# Autodesk Inventor assembly: ГОРИЗОНТАЛЬНЫЙ ЗАХВАТ 1 версия
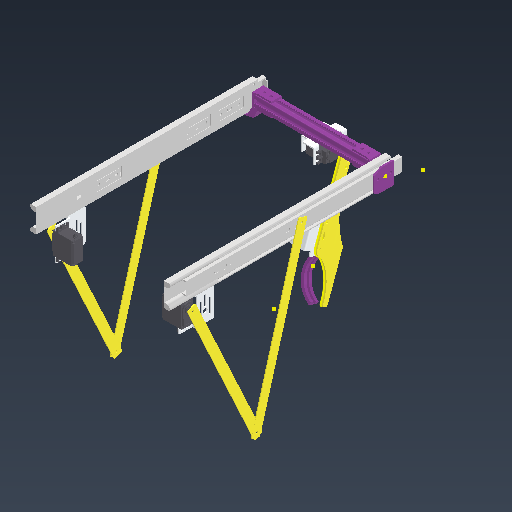
[picture p0: Inventor's stored thumbnail of the model, 512x512]
Saved by Autodesk Inventor 2025 (Build 290162000, 162)
## iProperties
Created: 2025-01-28
Part Number: ГОРИЗОНТАЛЬНЫЙ ЗАХВАТ 1 версия
Document SubType Name: Assembly
Designer: GameHD
Author: GameHD
## Documents named in this file (20)
- C:\Users\GameHD\Desktop\phantom 16950\ГОРИЗОНТАЛЬНЫЙ ЗАХВАТ 1 версия.iam
- C:\Users\GameHD\Desktop\phantom 16950\40 направляшка.iam
- C:\Users\GameHD\Desktop\phantom 16950\39070_TXM-288mm Flat Bar\39070_TXM-288mm Flat Bar.ipt
- C:\Users\GameHD\Desktop\phantom 16950\39280_txm-adjustableservobrackets\39280_txm-adjustableservobrackets.ipt
- C:\Users\GameHD\Desktop\phantom 16950\2000-0025-0002\2000-0025-0002.ipt
- C:\Users\GameHD\Desktop\phantom 16950\39070_TXM-288mm Flat Bar\длинная палка.ipt
- C:\Users\GameHD\Desktop\phantom 16950\39070_TXM-288mm Flat Bar\39070_TXM-288mm Flat Bar_MIR.ipt
- C:\Users\GameHD\Desktop\phantom 16950\39280_txm-adjustableservobrackets\39280_txm-adjustableservobrackets_MIR.ipt
- C:\Users\GameHD\Desktop\phantom 16950\2000-0025-0002\2000-0025-0002_MIR.ipt
- C:\Users\GameHD\Desktop\phantom 16950\39070_TXM-288mm Flat Bar\длинная палка_MIR.ipt
- C:\Users\GameHD\Desktop\phantom 16950\МЕЖДУ НАПРАВЛЯШКАМИ.ipt
- C:\Users\GameHD\Desktop\phantom 16950\39060_txm-standard servo bracket\39060_txm-standard servo bracket_MIR1.ipt
- C:\Users\GameHD\Desktop\phantom 16950\2000-0025-0002\2000-0025-0002_MIR2.ipt
- C:\Users\GameHD\Desktop\phantom 16950\DS3225_MG_metal_horn\DS3225_MG_metal_horn_MIR1.ipt
- C:\Users\GameHD\Desktop\phantom 16950\клешня сос_MIR1_MIR.ipt
- C:\Users\GameHD\Desktop\phantom 16950\39060_txm-standard servo bracket\39060_txm-standard servo bracket_MIR1_MIR.ipt
- C:\Users\GameHD\Desktop\phantom 16950\2000-0025-0002\2000-0025-0002_MIR2_MIR.ipt
- C:\Users\GameHD\Desktop\phantom 16950\Клешни с фиксатором\Клешни с фиксатором_MIR_MIR1_MIR.ipt
- C:\Users\GameHD\Desktop\phantom 16950\уголок п образный\уголок п образный.ipt
- C:\Users\GameHD\Desktop\phantom 16950\уголок п образный\уголок п образный_MIR.ipt
## Components (20 placed, 19 different names)
1. 40 направляшка:1 [sub-assembly]
2. 40 направляшка:2 [sub-assembly]
3. 39070_TXM-288mm Flat Bar:1
4. 39280_txm-adjustableservobrackets:1
5. 2000-0025-0002:1
6. длинная палка:1
7. 39070_TXM-288mm Flat Bar_MIR:1
8. 39280_txm-adjustableservobrackets_MIR:1
9. 2000-0025-0002_MIR:1
10. длинная палка_MIR:1
11. МЕЖДУ НАПРАВЛЯШКАМИ:1
12. 39060_txm-standard servo bracket_MIR1:1
13. 2000-0025-0002_MIR2:1
14. DS3225_MG_metal_horn_MIR1:1
15. клешня сос_MIR1_MIR:1
16. 39060_txm-standard servo bracket_MIR1_MIR:1
17. 2000-0025-0002_MIR2_MIR:1
18. Клешни с фиксатором_MIR_MIR1_MIR:1
19. уголок п образный:1
20. уголок п образный_MIR:1
## Relationships (42: Mate 33, Flush 9)
- [Mate]: 40 направляшка:1 ↔ 39280_txm-adjustableservobrackets:1
- [Mate]: 39280_txm-adjustableservobrackets:1 ↔ 2000-0025-0002:1
- [Mate]: 39280_txm-adjustableservobrackets:1 ↔ 2000-0025-0002:1
- [Mate]: 39070_TXM-288mm Flat Bar:1 ↔ 2000-0025-0002:1
- [Mate]: 39070_TXM-288mm Flat Bar:1 ↔ длинная палка:1
- [Mate]: 40 направляшка:1 ↔ длинная палка:1
- [Mate]: 39070_TXM-288mm Flat Bar_MIR:1 ↔ 2000-0025-0002_MIR:1
- [Mate]: 39280_txm-adjustableservobrackets_MIR:1 ↔ 2000-0025-0002_MIR:1
- [Mate]: 39280_txm-adjustableservobrackets_MIR:1 ↔ 2000-0025-0002_MIR:1
- [Mate]: 39070_TXM-288mm Flat Bar_MIR:1 ↔ длинная палка_MIR:1
- [Mate]: 39280_txm-adjustableservobrackets_MIR:1 ↔ 2000-0025-0002_MIR:1
- [Mate]: 39280_txm-adjustableservobrackets_MIR:1 ↔ 2000-0025-0002_MIR:1
- [Mate]: 40 направляшка:2 ↔ длинная палка_MIR:1
- [Mate]: 39060_txm-standard servo bracket_MIR1:1 ↔ 2000-0025-0002_MIR2:1
- [Mate] (1 mm): 2000-0025-0002_MIR2:1 ↔ DS3225_MG_metal_horn_MIR1:1
- [Mate]: 2000-0025-0002_MIR2:1 ↔ DS3225_MG_metal_horn_MIR1:1
- [Mate]: клешня сос_MIR1_MIR:1 ↔ 39060_txm-standard servo bracket_MIR1_MIR:1
- [Flush]: клешня сос_MIR1_MIR:1 ↔ 39060_txm-standard servo bracket_MIR1_MIR:1
- [Flush] (-90 mm): клешня сос_MIR1_MIR:1 ↔ 39060_txm-standard servo bracket_MIR1_MIR:1
- [Mate]: 39060_txm-standard servo bracket_MIR1_MIR:1 ↔ 2000-0025-0002_MIR2_MIR:1
- [Flush] (2.5 mm): 39060_txm-standard servo bracket_MIR1_MIR:1 ↔ 2000-0025-0002_MIR2_MIR:1
- [Mate] (4 mm): 39060_txm-standard servo bracket_MIR1_MIR:1 ↔ 2000-0025-0002_MIR2_MIR:1
- [Mate]: 2000-0025-0002_MIR2_MIR:1 ↔ Клешни с фиксатором_MIR_MIR1_MIR:1
- [Mate]: 2000-0025-0002_MIR2_MIR:1 ↔ Клешни с фиксатором_MIR_MIR1_MIR:1
- [Mate] (7 mm): клешня сос_MIR1_MIR:1 ↔ Клешни с фиксатором_MIR_MIR1_MIR:1
- [Mate]: DS3225_MG_metal_horn_MIR1:1 ↔ клешня сос_MIR1_MIR:1
- [Mate] (2.5 mm): DS3225_MG_metal_horn_MIR1:1 ↔ клешня сос_MIR1_MIR:1
- [Flush] (11.5 mm): DS3225_MG_metal_horn_MIR1:1 ↔ клешня сос_MIR1_MIR:1
- [Mate]: МЕЖДУ НАПРАВЛЯШКАМИ:1 ↔ 39060_txm-standard servo bracket_MIR1:1
- [Flush] (9.8 mm): МЕЖДУ НАПРАВЛЯШКАМИ:1 ↔ 39060_txm-standard servo bracket_MIR1:1
- [Mate] (4.5 mm): 39060_txm-standard servo bracket_MIR1:1 ↔ 2000-0025-0002_MIR2:1
- [Flush] (2 mm): 39060_txm-standard servo bracket_MIR1:1 ↔ 2000-0025-0002_MIR2:1
- [Mate]: 40 направляшка:2 ↔ уголок п образный:1
- [Mate]: 40 направляшка:2 ↔ уголок п образный:1
- [Mate]: МЕЖДУ НАПРАВЛЯШКАМИ:1 ↔ уголок п образный:1
- [Mate]: МЕЖДУ НАПРАВЛЯШКАМИ:1 ↔ уголок п образный:1
- [Flush]: МЕЖДУ НАПРАВЛЯШКАМИ:1 ↔ уголок п образный:1
- [Flush] (-18.5 mm): 40 направляшка:2 ↔ уголок п образный:1
- [Mate]: 40 направляшка:1 ↔ уголок п образный_MIR:1
- [Mate]: 40 направляшка:1 ↔ уголок п образный_MIR:1
- [Mate]: МЕЖДУ НАПРАВЛЯШКАМИ:1 ↔ уголок п образный_MIR:1
- [Flush]: уголок п образный:1 ↔ уголок п образный_MIR:1
